# Autodesk Inventor assembly: SUBLoadCellBase
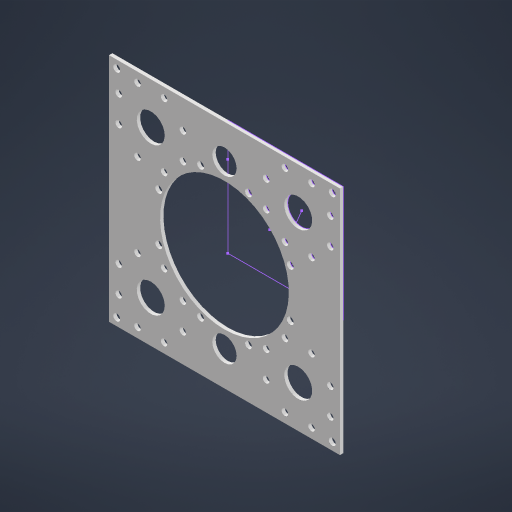
[picture p0: Inventor's stored thumbnail of the model, 512x512]
Saved by Autodesk Inventor 2024 (Build 280153000, 153)
## iProperties
Created: 2025-02-12
Part Number: SUBLoadCellBase
Document SubType Name: Assembly
Designer: Tommy Rohmann
Author: Tommy Rohmann
## Documents named in this file (3)
- C:\Users\Tommy Rohmann\OneDrive\Projects\Microgravity-Press-Washing-Machine\System Design and Documentation\Inventor Design Project\SUBLoadCellBase.iam
- C:\Users\Tommy Rohmann\OneDrive\Projects\Microgravity-Press-Washing-Machine\System Design and Documentation\Inventor Design Project\LAYOUT.ipt
- C:\Users\Tommy Rohmann\OneDrive\Projects\Microgravity-Press-Washing-Machine\System Design and Documentation\Inventor Design Project\MotorAndLoadCellBase.iam
## Components (2 placed, 2 different names)
1. LAYOUT:1
2. MotorAndLoadCellBase:1 [sub-assembly]
## Relationships (1: Composite 1)
- [Composite]: LAYOUT:1 ↔ MotorAndLoadCellBase:1
